# Autodesk Inventor assembly: LearningKitWindAlt
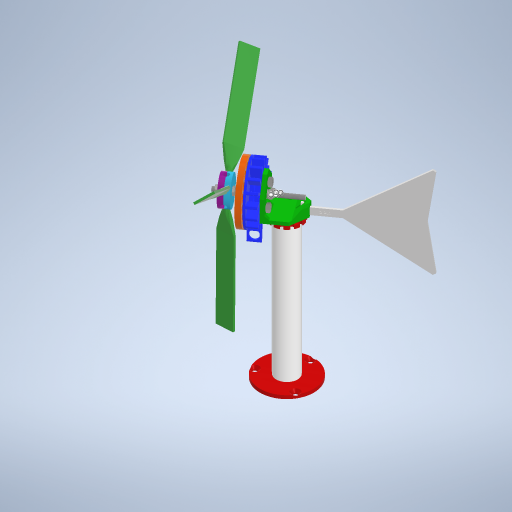
[picture p0: Inventor's stored thumbnail of the model, 512x512]
Saved by Autodesk Inventor 2024.3 (Build 283343000, 343)
## iProperties
Created: 2024-11-20
Part Number: LearningKitWindAlt
Document SubType Name: Assembly
Designer: Maximilian Hock
Author: Maximilian Hock
## Documents named in this file (10)
- Z:\Dokumente\LearningKit\LearningKitWind\LearningKitWind.iam
- Z:\Dokumente\LearningKit\LearningKitWind\WindFoot.ipt
- Z:\Dokumente\LearningKit\LearningKitWind\WindTowerNacelleInterface.ipt
- Z:\Dokumente\Inventor\Content Center Files\R2024\de-DE\SKF - Single row ball bearings\SKF608.ipt
- Z:\Dokumente\LearningKit\LearningKitWind\WindRotor.iam
- Z:\Dokumente\Inventor\Content Center Files\R2024\de-DE\DIN EN ISO 4032\DIN EN ISO 4032 - M6.ipt
- Z:\Dokumente\LearningKit\LearningKitGenerator\PancakeGenerator.iam
- Z:\Dokumente\LearningKit\LearningKitWind\WindTower.ipt
- Z:\Dokumente\LearningKit\LearningKitWind\WindNacelle.ipt
- Z:\Dokumente\LearningKit\LearningKitWind\WindFin.ipt
## Components (13 placed, 9 different names)
1. WindFoot:1 — Starr:12, Passend:1, Passend:2, Passend:3
2. WindTowerNacelleInterface:1 — Starr:10, Starr:13
3. WindRotor:1 [sub-assembly] — Zylindrisch:12, Planar:8, Drehbar:23
4. WindTower:1 — Starr:12, Starr:13
5. DIN EN ISO 4032 M6:1 — Drehbar:21
6. DIN EN ISO 4032 M6:2 — Drehbar:20
7. DIN EN ISO 4032 M6:3 — Drehbar:22
8. WindNacelle:1 — Zylindrisch:10, Zylindrisch:11, Drehbar:20, Drehbar:21, Drehbar:22, Drehbar:24, Planar:9, Starr:14
9. SKF- Kugellager, einreihig SKF608:3 — Starr:10, Starr:11
10. WindFin:1 — Starr:14
11. PancakeGenerator:1 [sub-assembly] — Zylindrisch:10, Zylindrisch:11, Zylindrisch:12, Planar:8, Planar:9
12. DIN EN ISO 4032 M6:6 — Drehbar:23
13. SKF- Kugellager, einreihig SKF608:4 — Starr:11, Drehbar:24
## Relationships (18: RevoluteJoint 5, WeldJoint 5, CylindricalJoint 3, Mate 3, PlanarJoint 2)
- Zylindrisch:10 [CylindricalJoint]: WindNacelle:1 ↔ PancakeGenerator:1
- Zylindrisch:11 [CylindricalJoint]: WindNacelle:1 ↔ PancakeGenerator:1
- Drehbar:20 [RevoluteJoint]: DIN EN ISO 4032 M6:2 ↔ WindNacelle:1
- Drehbar:21 [RevoluteJoint]: DIN EN ISO 4032 M6:1 ↔ WindNacelle:1
- Drehbar:22 [RevoluteJoint]: DIN EN ISO 4032 M6:3 ↔ WindNacelle:1
- Zylindrisch:12 [CylindricalJoint]: WindRotor:1 ↔ PancakeGenerator:1
- Planar:8: WindRotor:1 ↔ PancakeGenerator:1
- Drehbar:23 [RevoluteJoint]: WindRotor:1 ↔ DIN EN ISO 4032 M6:6
- Starr:10 [WeldJoint]: WindTowerNacelleInterface:1 ↔ SKF- Kugellager, einreihig SKF608:3
- Starr:11 [WeldJoint]: SKF- Kugellager, einreihig SKF608:3 ↔ SKF- Kugellager, einreihig SKF608:4
- Drehbar:24 [RevoluteJoint]: WindNacelle:1 ↔ SKF- Kugellager, einreihig SKF608:4
- Starr:12 [WeldJoint]: WindFoot:1 ↔ WindTower:1
- Starr:13 [WeldJoint]: WindTowerNacelleInterface:1 ↔ WindTower:1
- Passend:1 [Mate]: WindFoot:1
- Passend:2 [Mate]: WindFoot:1
- Passend:3 [Mate]: WindFoot:1
- Planar:9: WindNacelle:1 ↔ PancakeGenerator:1
- Starr:14 [WeldJoint]: WindNacelle:1 ↔ WindFin:1
